# Autodesk Inventor assembly: HighBatteryFront
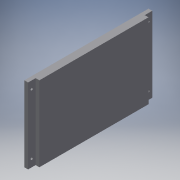
[picture p0: Inventor's stored thumbnail of the model, 180x180]
Saved by Autodesk Inventor 2019 (Build 230136000, 136)
## iProperties
Created: 2017-11-11
Part Number: HighBatteryFront
Document SubType Name: Assembly
Designer: james
Author: james
## Documents named in this file (4)
- F:\JimsDesign\2019CHS4089\HighBatteryFront.iam
- X:\Documents\Inventor\Jims2018CHS\BatteryHighFront.ipt
- X:\Documents\Inventor\Jims2018CHS\4089.ipt
- X:\Documents\Inventor\Jims2018CHS\Stealth.ipt
## Components (3 placed, 3 different names)
1. BatteryHighFront:1 — Mate:1, Mate:2
2. 4089:1 — Mate:2
3. Stealth:1 — Mate:1
## Relationships (2: Mate 2)
- Mate:1: BatteryHighFront:1 ↔ Stealth:1
- Mate:2: BatteryHighFront:1 ↔ 4089:1
